# Autodesk Inventor assembly: HbIndexFingerForChild
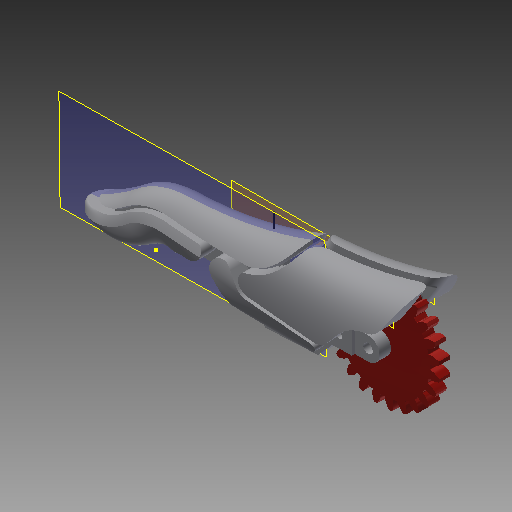
[picture p0: Inventor's stored thumbnail of the model, 512x512]
Saved by Autodesk Inventor 2017 (Build 210142000, 142)
## iProperties
Part Number: HbIndexFingerForChild
Material: 一般
Document SubType Name: Assembly
Designer: sktom
Author: sktom
## Documents named in this file (11)
- D:\OneDrive\CAD\MAJ\hackberry\HACKberry-hardware\3D_69%inlength\Inventor\HbHandForChild\HbIndexFinger01ForChild\HbIndexFinger01ForChild.iam
- D:\OneDrive\CAD\MAJ\hackberry\HACKberry-hardware\3D_69%inlength\Inventor\HbHandForChild\HbIndexFinger01ForChild\HbIndexInputLink02ForChild.ipt
- D:\OneDrive\CAD\MAJ\hackberry\HACKberry-hardware\3D_69%inlength\Inventor\HbHandForChild\HbIndexFinger01ForChild\HbIndexMiddle-DistalPhalanx02ForChild.ipt
- D:\OneDrive\CAD\MAJ\hackberry\HACKberry-hardware\3D_69%inlength\Inventor\HbHandForChild\HbIndexFinger01ForChild\HbIndexCouplerLink02ForChild.ipt
- D:\OneDrive\CAD\MAJ\hackberry\HACKberry-hardware\3D_69%inlength\Inventor\HbHandForChild\HbIndexFinger01ForChild\HbIndexCouplerLinkCover02ForChild.ipt
- D:\OneDrive\CAD\MAJ\hackberry\HACKberry-hardware\3D_69%inlength\Inventor\HbHandForChild\HbIndexFinger01ForChild\HbIndexProximalPhalanx03ForChild.ipt
- D:\OneDrive\CAD\MAJ\hackberry\HACKberry-hardware\3D_69%inlength\Inventor\HbHandForChild\HbIndexFinger01ForChild\HbIndexProximalPhalanxCover02ForChild.ipt
- D:\OneDrive\CAD\MAJ\hackberry\HACKberry-hardware\3D_69%inlength\Inventor\HbHandForChild\HbIndexFinger01ForChild\HbIndexReleaseLever02ForChild.ipt
- D:\OneDrive\CAD\MAJ\hackberry\HACKberry-hardware\3D_69%inlength\Inventor\HbHandForChild\HbIndexFinger01ForChild\Spur Gear (24 teeth).ipt
- D:\OneDrive\CAD\MAJ\hackberry\HACKberry-hardware\3D_69%inlength\Inventor\HbHandForChild\HbIndexFinger01ForChild\shaft_phi1.5_l6.ipt
- D:\OneDrive\CAD\MAJ\hackberry\HACKberry-hardware\3D_69%inlength\Inventor\HbHandForChild\TOS 0.3-3-270ﾟ-3.ipt
## Components (13 placed, 10 different names)
1. HbIndexInputLink02ForChild:1 — 挿入:4, 円柱状:1, 円柱状:3
2. HbIndexMiddle-DistalPhalanx02ForChild:1 — 挿入:1, 挿入:5, 円柱状:2
3. HbIndexCouplerLink02ForChild:1 — 挿入:1, 挿入:2, 挿入:3, 挿入:4, 挿入:12, 挿入:14
4. HbIndexCouplerLinkCover02ForChild:1 — 挿入:2, 挿入:3, 挿入:10
5. HbIndexProximalPhalanx03ForChild:1 — 円柱状:2, 円柱状:3, 挿入:9
6. HbIndexProximalPhalanxCover02ForChild:1 — 挿入:5, 円柱状:1, 挿入:8, 挿入:11, 挿入:13
7. HbIndexReleaseLever02ForChild:1 — 挿入:8
8. Spur Gear (24 teeth):1 — 挿入:9, 挿入:10
9. shaft_phi1.5_l6:1 — 挿入:11
10. shaft_phi1.5_l6:2 — 挿入:12
11. shaft_phi1.5_l6:3 — 挿入:13
12. shaft_phi1.5_l6:4 — 挿入:14
13. TOS 0.3-3-270ﾟ-3:1
## Relationships (15: Insert 12, CylindricalJoint 3)
- 挿入:1 [Insert] (0.4 mm): HbIndexMiddle-DistalPhalanx02ForChild:1 ↔ HbIndexCouplerLink02ForChild:1
- 挿入:2 [Insert]: HbIndexCouplerLink02ForChild:1 ↔ HbIndexCouplerLinkCover02ForChild:1
- 挿入:3 [Insert]: HbIndexCouplerLink02ForChild:1 ↔ HbIndexCouplerLinkCover02ForChild:1
- 挿入:4 [Insert] (0.25 mm): HbIndexInputLink02ForChild:1 ↔ HbIndexCouplerLink02ForChild:1
- 挿入:5 [Insert] (0.4 mm): HbIndexMiddle-DistalPhalanx02ForChild:1 ↔ HbIndexProximalPhalanxCover02ForChild:1
- 円柱状:1 [CylindricalJoint]: HbIndexInputLink02ForChild:1 ↔ HbIndexProximalPhalanxCover02ForChild:1
- 挿入:8 [Insert] (0.2 mm): HbIndexProximalPhalanxCover02ForChild:1 ↔ HbIndexReleaseLever02ForChild:1
- 円柱状:2 [CylindricalJoint]: HbIndexMiddle-DistalPhalanx02ForChild:1 ↔ HbIndexProximalPhalanx03ForChild:1
- 円柱状:3 [CylindricalJoint]: HbIndexInputLink02ForChild:1 ↔ HbIndexProximalPhalanx03ForChild:1
- 挿入:9 [Insert]: HbIndexProximalPhalanx03ForChild:1 ↔ Spur Gear (24 teeth):1
- 挿入:10 [Insert]: HbIndexCouplerLinkCover02ForChild:1 ↔ Spur Gear (24 teeth):1
- 挿入:11 [Insert] (0.5 mm): HbIndexProximalPhalanxCover02ForChild:1 ↔ shaft_phi1.5_l6:1
- 挿入:12 [Insert] (0.5 mm): HbIndexCouplerLink02ForChild:1 ↔ shaft_phi1.5_l6:2
- 挿入:13 [Insert] (0.5 mm): HbIndexProximalPhalanxCover02ForChild:1 ↔ shaft_phi1.5_l6:3
- 挿入:14 [Insert] (-2 mm): HbIndexCouplerLink02ForChild:1 ↔ shaft_phi1.5_l6:4
